# Autodesk Inventor assembly: Assembly_motorcoverbase
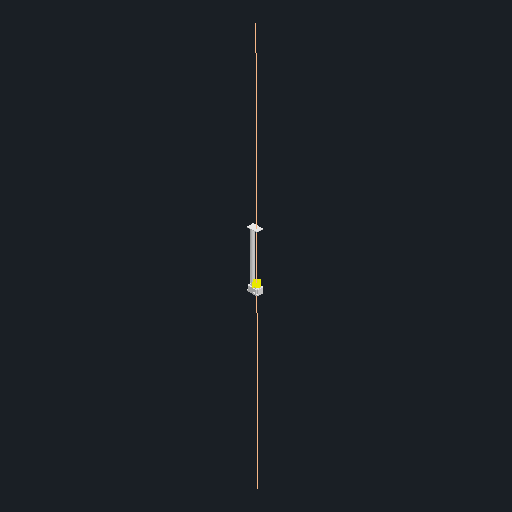
[picture p0: Inventor's stored thumbnail of the model, 512x512]
Saved by Autodesk Inventor 2024.2 (Build 282272000, 272)
## iProperties
Created: 2024-03-21
Part Number: Assembly_motorcoverbase
Document SubType Name: Assembly
Designer: seifs
Author: seifs
## Documents named in this file (11)
- C:\Users\seifs\Downloads\Final Assembly\Assembly_motorcoverbase_2.iam
- C:\Users\seifs\Downloads\Final Assembly\project_base.ipt
- C:\Users\seifs\Downloads\Final Assembly\NEMA17 Stepper Motor.ipt
- C:\Users\seifs\Downloads\Final Assembly\motor_cover_final.ipt
- C:\Users\seifs\Downloads\Final Assembly\pvc.ipt
- C:\Users\seifs\Downloads\Final Assembly\coupler.ipt
- C:\Users\seifs\Downloads\Final Assembly\LeadScrew1.ipt
- C:\Users\seifs\Downloads\Final Assembly\Top_part.ipt
- C:\Users\seifs\OneDrive\Documents\Inventor\Content Center Files\R2024\en-US\Bearing GB_T 292-2007\Rolling bearing B708 C GB_T 292-2007.ipt
- C:\Users\seifs\Downloads\Final Assembly\ISO 7046-1 - M3 x 16_ - 4.8 - Z - ISO.ipt
- C:\Users\seifs\Downloads\Final Assembly\ISO 4036 - M3(2).ipt
## Components (20 placed, 10 different names)
1. project_base:1 — Insert:1, Insert:2, Insert:5, Insert:28, Insert:29, Insert:30, Insert:31
2. motor_cover_final:1 — Insert:1, Insert:2, Insert:3, Insert:4, Insert:12, Insert:13, Insert:14, Insert:15, Insert:16, Insert:17, Insert:18, Insert:19
3. NEMA17 Stepper Motor:1 — Insert:3, Insert:4, Insert:6
4. pvc:1 — Insert:5, Flush:1
5. coupler:1 — Insert:6, Insert:10
6. LeadScrew1:1 — Insert:10
7. Top_part:1 — Flush:1, Insert:11
8. Bearing GB/T 292-2007 Type IN - withdrawn B708 C:1 — Insert:11
9. ISO 7046-1 Z M3 x 16 - 4.8 - Z:1 — Insert:12
10. ISO 7046-1 Z M3 x 16 - 4.8 - Z:2 — Insert:15
11. ISO 7046-1 Z M3 x 16 - 4.8 - Z:3 — Insert:14
12. ISO 7046-1 Z M3 x 16 - 4.8 - Z:4 — Insert:13
13. ISO 7046-1 Z M3 x 16 - 4.8 - Z:5 — Insert:16
14. ISO 7046-1 Z M3 x 16 - 4.8 - Z:6 — Insert:17
15. ISO 7046-1 Z M3 x 16 - 4.8 - Z:7 — Insert:18
16. ISO 7046-1 Z M3 x 16 - 4.8 - Z:8 — Insert:19
17. ISO 4036 M3:5 — Insert:31
18. ISO 4036 M3:6 — Insert:29
19. ISO 4036 M3:7 — Insert:30
20. ISO 4036 M3:8 — Insert:28
## Relationships (21: Insert 20, Flush 1)
- Insert:1: project_base:1 ↔ motor_cover_final:1
- Insert:2: project_base:1 ↔ motor_cover_final:1
- Insert:3: motor_cover_final:1 ↔ NEMA17 Stepper Motor:1
- Insert:4: motor_cover_final:1 ↔ NEMA17 Stepper Motor:1
- Insert:5: project_base:1 ↔ pvc:1
- Insert:6 (-15 mm): NEMA17 Stepper Motor:1 ↔ coupler:1
- Insert:10 (-8 mm): coupler:1 ↔ LeadScrew1:1
- Flush:1: pvc:1 ↔ Top_part:1
- Insert:11: Top_part:1 ↔ Bearing GB/T 292-2007 Type IN - withdrawn B708 C:1
- Insert:12: motor_cover_final:1 ↔ ISO 7046-1 Z M3 x 16 - 4.8 - Z:1
- Insert:13: motor_cover_final:1 ↔ ISO 7046-1 Z M3 x 16 - 4.8 - Z:4
- Insert:14: motor_cover_final:1 ↔ ISO 7046-1 Z M3 x 16 - 4.8 - Z:3
- Insert:15: motor_cover_final:1 ↔ ISO 7046-1 Z M3 x 16 - 4.8 - Z:2
- Insert:16: motor_cover_final:1 ↔ ISO 7046-1 Z M3 x 16 - 4.8 - Z:5
- Insert:17: motor_cover_final:1 ↔ ISO 7046-1 Z M3 x 16 - 4.8 - Z:6
- Insert:18: motor_cover_final:1 ↔ ISO 7046-1 Z M3 x 16 - 4.8 - Z:7
- Insert:19: motor_cover_final:1 ↔ ISO 7046-1 Z M3 x 16 - 4.8 - Z:8
- Insert:28: project_base:1 ↔ ISO 4036 M3:8
- Insert:29: project_base:1 ↔ ISO 4036 M3:6
- Insert:30: project_base:1 ↔ ISO 4036 M3:7
- Insert:31: project_base:1 ↔ ISO 4036 M3:5
